# Autodesk Inventor assembly: montagemEstruturaCameraCME
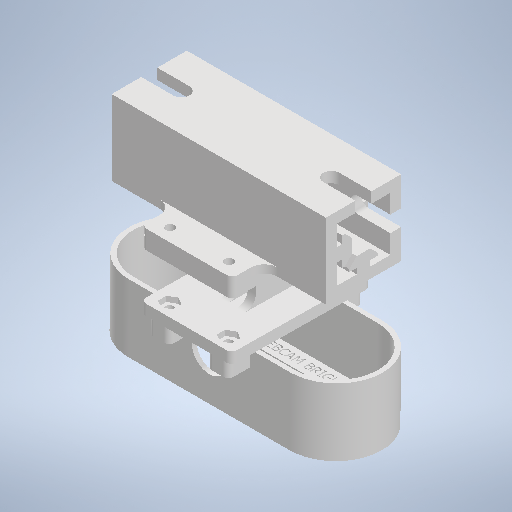
[picture p0: Inventor's stored thumbnail of the model, 512x512]
Saved by Autodesk Inventor 2025 (Build 290162000, 162)
## iProperties
Created: 2024-04-10
Part Number: montagemEstruturaCameraCME
Document SubType Name: Assembly
Designer: cvss2
Author: cvss2
## Documents named in this file (4)
- C:\Users\cvss2.CINSOFTEX\Documents\GitHub\CME-3d-models\Estrutura Camera CME - Copy\montagemEstruturaCameraCME.iam
- C:\Users\cvss2.CINSOFTEX\Documents\GitHub\CME-3d-models\suporteBright2k.ipt
- C:\Users\cvss2.CINSOFTEX\Documents\GitHub\CME-3d-models\Estrutura Camera CME - Copy\cameraSlider.ipt
- C:\Users\cvss2.CINSOFTEX\Documents\GitHub\CME-3d-models\Estrutura Camera CME - Copy\encaixeDuplo.ipt
## Components (4 placed, 3 different names)
1. cameraSlider:2 — Mate:33, Mate:34, Mate:35
2. encaixeDuplo:1 — Mate:29, Mate:30, Mate:33, Mate:34, Mate:35
3. encaixeDuplo:2 — Mate:29, Mate:30, Mate:36, Mate:37, Mate:38
4. suporteBright2k:2 — Mate:36, Mate:37, Mate:38
## Relationships (8: Mate 8)
- Mate:29: encaixeDuplo:1 ↔ encaixeDuplo:2
- Mate:30 (0.1 mm): encaixeDuplo:1 ↔ encaixeDuplo:2
- Mate:33: cameraSlider:2 ↔ encaixeDuplo:1
- Mate:34: cameraSlider:2 ↔ encaixeDuplo:1
- Mate:35: cameraSlider:2 ↔ encaixeDuplo:1
- Mate:36: encaixeDuplo:2 ↔ suporteBright2k:2
- Mate:37: encaixeDuplo:2 ↔ suporteBright2k:2
- Mate:38: encaixeDuplo:2 ↔ suporteBright2k:2
